# Autodesk Inventor assembly: Tuere
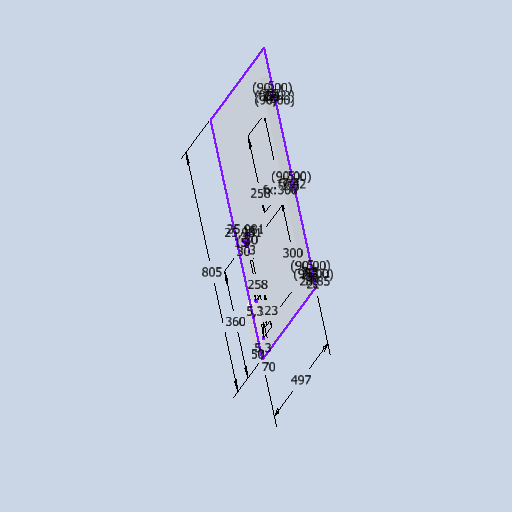
[picture p0: Inventor's stored thumbnail of the model, 512x512]
Saved by Autodesk Inventor 2022 (Build 260153000, 153)
## iProperties
Created: 2021-06-13
Part Number: Tuere
Document SubType Name: Assembly
Designer: Cornee
Author: Cornee
## Documents named in this file (8)
- C:\Users\kaebi\Desktop\07-CAD Files\06-Gesamtanlage\100_ZB_Gesamtanlage\Tuere\Tuere.iam
- C:\Users\kaebi\Desktop\07-CAD Files\06-Gesamtanlage\100_ZB_Gesamtanlage\Tuere\Plexiglas_Einfassung_Tuere.ipt
- C:\Users\kaebi\Desktop\07-CAD Files\06-Gesamtanlage\100_ZB_Gesamtanlage\Tuere\A_138x52x22_5mm_2009851_B.ipt
- C:\Users\kaebi\Desktop\07-CAD Files\06-Gesamtanlage\100_ZB_Gesamtanlage\Tuere\TuerHalter.ipt
- C:\Users\kaebi\Desktop\07-CAD Files\06-Gesamtanlage\100_ZB_Gesamtanlage\Tuere\Hinge1.ipt
- C:\Users\kaebi\Desktop\07-CAD Files\06-Gesamtanlage\100_ZB_Gesamtanlage\Tuere\Hinge2.ipt
- C:\Users\kaebi\Desktop\07-CAD Files\06-Gesamtanlage\100_ZB_Gesamtanlage\Tuere\Griff_Ring.ipt
- C:\Users\kaebi\Desktop\07-CAD Files\06-Gesamtanlage\100_ZB_Gesamtanlage\Tuere\Griff_Deckel.ipt
## Components (13 placed, 7 different names)
1. Plexiglas_Einfassung_Tuere:1 — Mate:1, Flush:1, Mate:2, Mate:50, Mate:52, Angle:1, Mate:65, Mate:66, Mate:67, Mate:68, Mate:69, Mate:70, Mate:71
2. A_138x52x22_5mm_2009851_B:1 — Mate:1, Flush:1, Mate:2
3. TuerHalter:1 — Mate:23, Mate:24, Mate:33, Flush:3, Flush:4, Flush:5, Mate:34, Mate:35, Mate:36, Mate:37, Mate:38, Mate:39, Mate:60
4. Hinge1:1 — Rotational:1, Flush:5, Mate:38, Mate:39, Mate:60
5. Hinge1:2 — Rotational:2, Mate:24, Flush:4, Mate:36, Mate:37, Angle:1
6. Hinge1:3 — Rotational:3, Mate:23, Mate:33, Flush:3, Mate:34, Mate:35
7. Hinge2:1 — Rotational:1, Mate:69, Mate:70, Mate:71
8. Hinge2:2 — Rotational:2, Mate:65
9. Hinge2:3 — Rotational:3, Mate:66, Mate:67, Mate:68
10. Griff_Ring:1 — Mate:42, Mate:43, Mate:56, Mate:57, Mate:58, Mate:59
11. Griff_Ring:2 — Mate:43, Mate:51, Mate:54, Mate:55, Mate:56, Mate:57
12. Griff_Deckel:1 — Mate:42, Mate:58, Mate:59
13. Griff_Ring:3 — Mate:50, Mate:51, Mate:52, Mate:54, Mate:55
## Relationships (38: Mate 30, Flush 4, RevoluteJoint 3, Angle 1)
- Mate:1: Plexiglas_Einfassung_Tuere:1 ↔ A_138x52x22_5mm_2009851_B:1
- Flush:1 (5 mm): Plexiglas_Einfassung_Tuere:1 ↔ A_138x52x22_5mm_2009851_B:1
- Mate:2 (2.65 mm): Plexiglas_Einfassung_Tuere:1 ↔ A_138x52x22_5mm_2009851_B:1
- Rotational:1 [RevoluteJoint] (0.1 mm): Hinge1:1 ↔ Hinge2:1
- Rotational:2 [RevoluteJoint] (0.1 mm): Hinge1:2 ↔ Hinge2:2
- Rotational:3 [RevoluteJoint] (0.1 mm): Hinge1:3 ↔ Hinge2:3
- Mate:23: TuerHalter:1 ↔ Hinge1:3
- Mate:24: TuerHalter:1 ↔ Hinge1:2
- Mate:33 (7 mm): TuerHalter:1 ↔ Hinge1:3
- Flush:3: TuerHalter:1 ↔ Hinge1:3
- Flush:4: TuerHalter:1 ↔ Hinge1:2
- Flush:5: TuerHalter:1 ↔ Hinge1:1
- Mate:34 (7 mm): TuerHalter:1 ↔ Hinge1:3
- Mate:35 (7 mm): TuerHalter:1 ↔ Hinge1:3
- Mate:36 (7 mm): TuerHalter:1 ↔ Hinge1:2
- Mate:37 (7 mm): TuerHalter:1 ↔ Hinge1:2
- Mate:38 (7 mm): TuerHalter:1 ↔ Hinge1:1
- Mate:39 (7 mm): TuerHalter:1 ↔ Hinge1:1
- Mate:42: Griff_Ring:1 ↔ Griff_Deckel:1
- Mate:43: Griff_Ring:1 ↔ Griff_Ring:2
- Mate:50: Plexiglas_Einfassung_Tuere:1 ↔ Griff_Ring:3
- Mate:51: Griff_Ring:2 ↔ Griff_Ring:3
- Mate:52: Plexiglas_Einfassung_Tuere:1 ↔ Griff_Ring:3
- Mate:54: Griff_Ring:2 ↔ Griff_Ring:3
- Mate:55: Griff_Ring:2 ↔ Griff_Ring:3
- Mate:56: Griff_Ring:1 ↔ Griff_Ring:2
- Mate:57: Griff_Ring:1 ↔ Griff_Ring:2
- Mate:58: Griff_Ring:1 ↔ Griff_Deckel:1
- Mate:59: Griff_Ring:1 ↔ Griff_Deckel:1
- Mate:60: TuerHalter:1 ↔ Hinge1:1
- Angle:1 (270 deg): Plexiglas_Einfassung_Tuere:1 ↔ Hinge1:2
- Mate:65: Plexiglas_Einfassung_Tuere:1 ↔ Hinge2:2
- Mate:66: Plexiglas_Einfassung_Tuere:1 ↔ Hinge2:3
- Mate:67 (2.6 mm): Plexiglas_Einfassung_Tuere:1 ↔ Hinge2:3
- Mate:68 (2.6 mm): Plexiglas_Einfassung_Tuere:1 ↔ Hinge2:3
- Mate:69 (2.6 mm): Plexiglas_Einfassung_Tuere:1 ↔ Hinge2:1
- Mate:70 (2.6 mm): Plexiglas_Einfassung_Tuere:1 ↔ Hinge2:1
- Mate:71: Plexiglas_Einfassung_Tuere:1 ↔ Hinge2:1
